# Autodesk Inventor assembly: 15_1
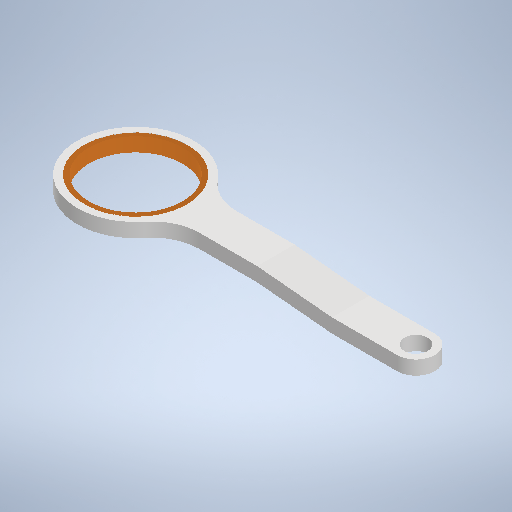
[picture p0: Inventor's stored thumbnail of the model, 512x512]
Saved by Autodesk Inventor 2025.1 (Build 291241000, 241)
## iProperties
Created: 2024-09-19
Part Number: 15_1
Document SubType Name: Assembly
Designer: ffogue
Author: ffogue
## Documents named in this file (3)
- C:\Users\ffogue\Documents\Inventor\Cylinder Radial Steam Engine\15_1.iam
- C:\Users\ffogue\Documents\Inventor\Cylinder Radial Steam Engine\15B.ipt
- C:\Users\ffogue\Documents\Inventor\Cylinder Radial Steam Engine\15fitting.ipt
## Components (2 placed, 2 different names)
1. 15B:1 — Mate:1, Flush:1
2. 15fitting:1 — Mate:1, Flush:1
## Relationships (2: Mate 1, Flush 1)
- Mate:1: 15B:1 ↔ 15fitting:1
- Flush:1: 15B:1 ↔ 15fitting:1
